# Autodesk Inventor assembly: Assembly1
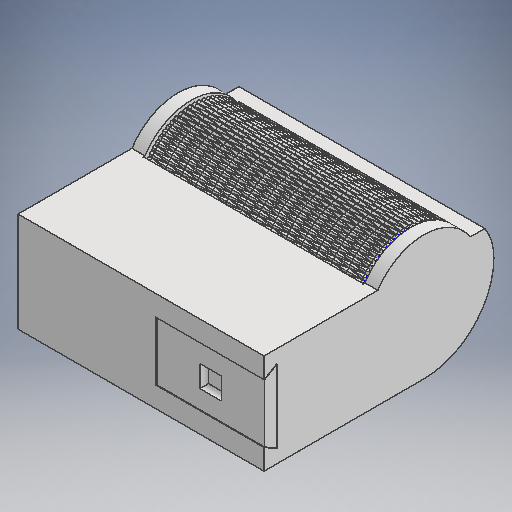
[picture p0: Inventor's stored thumbnail of the model, 512x512]
Saved by Autodesk Inventor 2025.2 (Build 292293000, 293)
## iProperties
Created: 2025-03-09
Part Number: Assembly1
Document SubType Name: Assembly
Designer: Alex
Author: Alex
## Documents named in this file (4)
- C:\Shared\alex-bartella-schoolwork\4b03\a1\a1.2\Assembly1.iam
- C:\Shared\alex-bartella-schoolwork\4b03\a1\a1.2\body.ipt
- C:\Shared\alex-bartella-schoolwork\4b03\a1\a1.2\roller.ipt
- C:\Shared\alex-bartella-schoolwork\4b03\a1\a1.1\door.ipt
## Components (3 placed, 3 different names)
1. body:1 — Mate:1, Mate:2, Mate:3, Flush:1, Mate:4, Flush:2
2. roller:1 — Mate:2, Mate:3
3. door:1 — Flush:1, Mate:4, Flush:2
## Relationships (6: Mate 4, Flush 2)
- Mate:1: body:1
- Mate:2: body:1 ↔ roller:1
- Mate:3 (0.3 mm): body:1 ↔ roller:1
- Flush:1 (0.1 mm): body:1 ↔ door:1
- Mate:4 (0.1 mm): body:1 ↔ door:1
- Flush:2: body:1 ↔ door:1
